# Autodesk Inventor assembly: дно
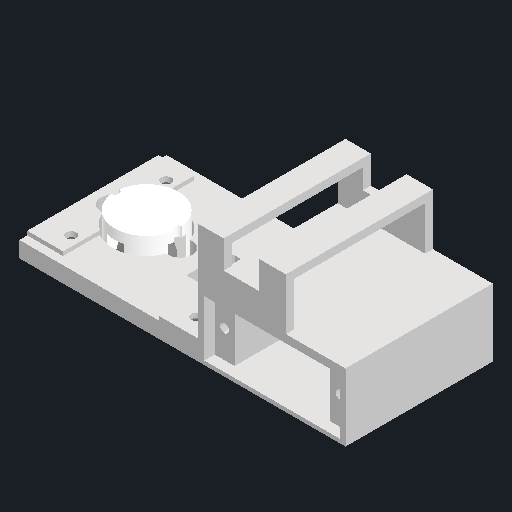
[picture p0: Inventor's stored thumbnail of the model, 512x512]
Saved by Autodesk Inventor 2022 (Build 260153000, 153)
## iProperties
Created: 2025-02-01
Part Number: дно
Document SubType Name: Assembly
Designer: it
Author: it
## Documents named in this file (4)
- E:\машина\дно.iam
- E:\машина\дно2.ipt
- C:\Users\it\Documents\Inventor\Content Center Files\R2022\ru-RU\Nut 3 GOST 15526-70\Гайка 3 M3 ГОСТ 15526-70.ipt
- E:\abuyz lkz vfibyrb\сфер.подшип.iam
## Components (6 placed, 3 different names)
1. дно2:1
2. Гайка 3 ГОСТ 15526-70 M3:1
3. Гайка 3 ГОСТ 15526-70 M3:2
4. Гайка 3 ГОСТ 15526-70 M3:3
5. Гайка 3 ГОСТ 15526-70 M3:4
6. сферич.подш:1 [sub-assembly]
## Relationships (9: Flush 5, Mate 4)
- [Flush]: дно2:1 ↔ Гайка 3 ГОСТ 15526-70 M3:3
- [Mate]: дно2:1 ↔ Гайка 3 ГОСТ 15526-70 M3:1
- [Flush]: дно2:1 ↔ Гайка 3 ГОСТ 15526-70 M3:1
- [Mate]: дно2:1 ↔ Гайка 3 ГОСТ 15526-70 M3:4
- [Flush]: дно2:1 ↔ Гайка 3 ГОСТ 15526-70 M3:2
- [Flush]: дно2:1 ↔ Гайка 3 ГОСТ 15526-70 M3:4
- [Flush]: дно2:1 ↔ Гайка 3 ГОСТ 15526-70 M3:2
- [Mate]: дно2:1 ↔ сферич.подш:1
- [Mate] (5.5235 mm): дно2:1 ↔ сферич.подш:1
